# Autodesk Inventor assembly: Connect
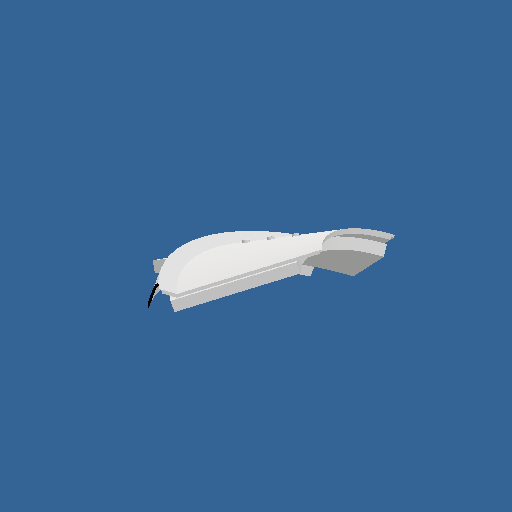
[picture p0: Inventor's stored thumbnail of the model, 512x512]
Saved by Autodesk Inventor 2026.2 (Build 302298000, 298)
## iProperties
Created: 2025-12-16
Part Number: Connect
Document SubType Name: Assembly
Designer: Thoma
Author: Thoma
## Documents named in this file (3)
- C:\Users\Thoma\OneDrive\Desktop\dir\telescope_cover\cover\Cover_Connect_Upper.iam
- C:\Users\Thoma\OneDrive\Desktop\dir\telescope_cover\cover\Cover_Upper_v2.ipt
- C:\Users\Thoma\OneDrive\Desktop\dir\telescope_cover\telescope\version_3\rod.ipt
## Components (2 placed, 2 different names)
1. Cover_Upper_v2:2 — Flush:3, Flush:4
2. rod:1 — Flush:3, Flush:4
## Relationships (2: Flush 2)
- Flush:3: Cover_Upper_v2:2 ↔ rod:1
- Flush:4: Cover_Upper_v2:2 ↔ rod:1
